# Autodesk Inventor assembly: Chassisv1
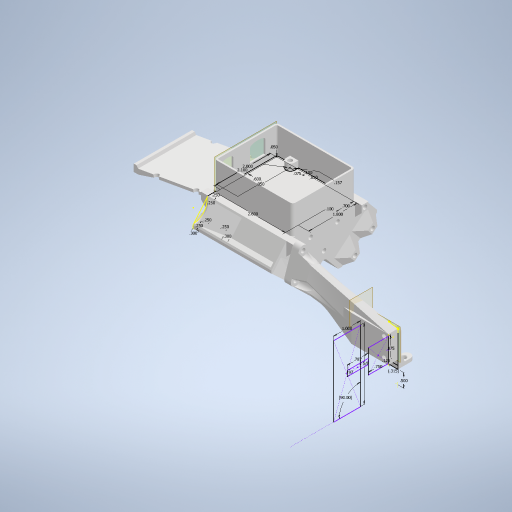
[picture p0: Inventor's stored thumbnail of the model, 512x512]
Saved by Autodesk Inventor 2024 (Build 280153020, 153B)
## iProperties
Created: 2024-03-25
Part Number: Chassisv1
Document SubType Name: Assembly
Designer: lvrectanus0
Author: lvrectanus0
## Documents named in this file (6)
- C:\Users\lvrectanus0\Documents\Github\SPARKLabs-ArduinoProjects\project\CAD\Autodesk\Chassisv1.iam
- C:\Users\lvrectanus0\Documents\Github\SPARKLabs-ArduinoProjects\project\CAD\Autodesk\ArduinoHolder-v2.ipt
- C:\Users\lvrectanus0\Documents\Github\SPARKLabs-ArduinoProjects\project\CAD\Autodesk\BatteryMount-v1.ipt
- C:\Users\lvrectanus0\Documents\Github\SPARKLabs-ArduinoProjects\project\CAD\Autodesk\BreadboardHolderv1.ipt
- C:\Users\lvrectanus0\Documents\Github\SPARKLabs-ArduinoProjects\project\CAD\Autodesk\Exports\MotorController-v1.ipt
- C:\Users\lvrectanus0\Documents\Sensor Mount.ipt
## Components (5 placed, 5 different names)
1. ArduinoHolder-v2:1 — Flush:1, Flush:2
2. BatteryMount-v1:1 — Flush:1, Flush:2, Flush:3, Flush:4
3. BreadboardHolderv1:1 — Flush:3
4. MotorController-v1:1 — Flush:4, Flush:5, Flush:6
5. Sensor Mount:1 — Flush:5, Flush:6
## Relationships (6: Flush 6)
- Flush:1: ArduinoHolder-v2:1 ↔ BatteryMount-v1:1
- Flush:2: ArduinoHolder-v2:1 ↔ BatteryMount-v1:1
- Flush:3: BatteryMount-v1:1 ↔ BreadboardHolderv1:1
- Flush:4: BatteryMount-v1:1 ↔ MotorController-v1:1
- Flush:5: MotorController-v1:1 ↔ Sensor Mount:1
- Flush:6: MotorController-v1:1 ↔ Sensor Mount:1
